# Autodesk Inventor assembly: PEMould_BaseAssembly
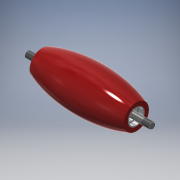
[picture p0: Inventor's stored thumbnail of the model, 180x180]
Saved by Autodesk Inventor 2018 (Build 220112000, 112)
## iProperties
Created: 2017-09-12
Part Number: PEMould_BaseAssembly
Document SubType Name: Assembly
Designer: P136265
Author: P136265
## Documents named in this file (4)
- C:\Users\P136265\Documents\mecanum-cad\PEMould_BaseAssembly.iam
- C:\Users\P136265\Documents\mecanum-cad\roller 8-19-6 bearing.ipt
- C:\Users\P136265\Documents\mecanum-cad\PE_Sleeve.ipt
- C:\Users\P136265\Documents\mecanum-cad\MecanumShaft.ipt
## Components (3 placed, 3 different names)
1. roller 8-19-6 bearing:1 — Angle:1, Mate:2, Mate:3, Mate:4, Mate:5, Mate:6, Angle:3, Mate:7
2. PE_Sleeve:1 — Mate:5, Mate:6
3. MecanumShaft:1 — Angle:1, Mate:2, Mate:3, Angle:2
## Relationships (9: Mate 6, Angle 3)
- Angle:1 (0 deg): roller 8-19-6 bearing:1 ↔ MecanumShaft:1
- Mate:2: roller 8-19-6 bearing:1 ↔ MecanumShaft:1
- Mate:3 (-25 mm): roller 8-19-6 bearing:1 ↔ MecanumShaft:1
- Mate:4: roller 8-19-6 bearing:1
- Angle:2 (0 deg): MecanumShaft:1
- Mate:5: roller 8-19-6 bearing:1 ↔ PE_Sleeve:1
- Mate:6: roller 8-19-6 bearing:1 ↔ PE_Sleeve:1
- Angle:3 (0 deg): roller 8-19-6 bearing:1
- Mate:7: roller 8-19-6 bearing:1
